# Autodesk Inventor assembly: Laser Galvo Module Assembly
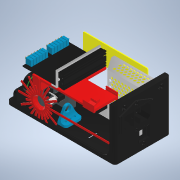
[picture p0: Inventor's stored thumbnail of the model, 180x180]
Saved by Autodesk Inventor 2021 (Build 250183000, 183)
## iProperties
Created: 2021-04-06
Part Number: Laser Galvo Module Assembly
Document SubType Name: Assembly
Designer: Andrew
Author: Andrew
## Documents named in this file (7)
- D:\Projects\acoustic_laser\cad\Laser Galvo Module Assembly.iam
- D:\Projects\acoustic_laser\cad\Control Board.ipt
- D:\Projects\acoustic_laser\cad\Laser Galvo Assembly.iam
- D:\Projects\acoustic_laser\cad\Power Supply.ipt
- D:\Projects\acoustic_laser\cad\Mount Plate.ipt
- D:\Projects\acoustic_laser\cad\Laser.ipt
- D:\Projects\acoustic_laser\cad\AC-14-F16A.ipt
## Components (7 placed, 6 different names)
1. Control Board:1
2. Laser Galvo Assembly:1 [sub-assembly] — Mate:3, Mate:7, Mate:8
3. Power Supply:1 — Mate:1, Mate:4, Mate:5
4. Mount Plate:1 — Flush:1, Flush:2, Flush:3, Mate:1, Mate:3, Mate:4, Mate:5, Mate:7, Mate:8, Mate:11, Mate:12, Mate:13, Mate:14, Flush:6, Flush:7, Mate:15, Flush:8, Flush:9
5. Laser:1 — Mate:11, Mate:12, Mate:13
6. AC-14-F16A:1 — Mate:14, Flush:6, Flush:7
7. Control Board:2 — Mate:15, Flush:8, Flush:9
## Relationships (18: Mate 11, Flush 7)
- Flush:1: Mount Plate:1
- Flush:2: Mount Plate:1
- Flush:3: Mount Plate:1
- Mate:1: Power Supply:1 ↔ Mount Plate:1
- Mate:3: Laser Galvo Assembly:1 ↔ Mount Plate:1
- Mate:4: Power Supply:1 ↔ Mount Plate:1
- Mate:5: Power Supply:1 ↔ Mount Plate:1
- Mate:7: Laser Galvo Assembly:1 ↔ Mount Plate:1
- Mate:8: Laser Galvo Assembly:1 ↔ Mount Plate:1
- Mate:11: Mount Plate:1 ↔ Laser:1
- Mate:12: Mount Plate:1 ↔ Laser:1
- Mate:13: Mount Plate:1 ↔ Laser:1
- Mate:14: Mount Plate:1 ↔ AC-14-F16A:1
- Flush:6 (12.5 mm): Mount Plate:1 ↔ AC-14-F16A:1
- Flush:7 (17.5 mm): Mount Plate:1 ↔ AC-14-F16A:1
- Mate:15: Mount Plate:1 ↔ Control Board:2
- Flush:8: Mount Plate:1 ↔ Control Board:2
- Flush:9: Mount Plate:1 ↔ Control Board:2
